# Autodesk Inventor assembly: КВ33.044.200
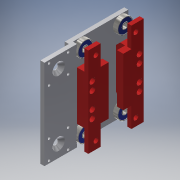
[picture p0: Inventor's stored thumbnail of the model, 180x180]
Saved by Autodesk Inventor 2019 (Build 230136000, 136)
## iProperties
Created: 2019-07-15
Part Number: КВ33.044.200
Material: Типовые
Document SubType Name: Assembly
Designer: Петров Иван
Description: Каретка оси Х
Author: Петров Иван
## Documents named in this file (4)
- C:\Users\user\Desktop\kvantoriada\kvantoriada\КВ33.044 - Оптимальный захват\КВ33.044.200 - Каретка оси Х.iam
- C:\Users\user\Desktop\kvantoriada\kvantoriada\КВ33.044 - Оптимальный захват\Стандартные изделия\Подшипник 626Z.ipt
- C:\Users\user\Desktop\kvantoriada\kvantoriada\КВ33.044 - Оптимальный захват\КВ33.044.202 - Фиксатор каретки.ipt
- C:\Users\user\Desktop\kvantoriada\kvantoriada\КВ33.044 - Оптимальный захват\КВ33.044.201 - Щека каретки.ipt
## Components (7 placed, 3 different names)
1. КВ33.044.201 - Щека каретки:1 — С поворотом:1, С поворотом:2, С поворотом:3, С поворотом:4, Жесткий:1, Жесткий:2
2. Подшипник 626Z:1 — С поворотом:1
3. Подшипник 626Z:2 — С поворотом:2
4. Подшипник 626Z:3 — С поворотом:3
5. Подшипник 626Z:4 — С поворотом:4
6. КВ33.044.202 - Фиксатор каретки:1 — Жесткий:1
7. КВ33.044.202 - Фиксатор каретки:2 — Жесткий:2
## Relationships (6: RevoluteJoint 4, WeldJoint 2)
- С поворотом:1 [RevoluteJoint]: КВ33.044.201 - Щека каретки:1 ↔ Подшипник 626Z:1
- С поворотом:2 [RevoluteJoint]: КВ33.044.201 - Щека каретки:1 ↔ Подшипник 626Z:2
- С поворотом:3 [RevoluteJoint]: КВ33.044.201 - Щека каретки:1 ↔ Подшипник 626Z:3
- С поворотом:4 [RevoluteJoint]: КВ33.044.201 - Щека каретки:1 ↔ Подшипник 626Z:4
- Жесткий:1 [WeldJoint]: КВ33.044.201 - Щека каретки:1 ↔ КВ33.044.202 - Фиксатор каретки:1
- Жесткий:2 [WeldJoint]: КВ33.044.201 - Щека каретки:1 ↔ КВ33.044.202 - Фиксатор каретки:2
